# Autodesk Inventor assembly: Wheels_hubs
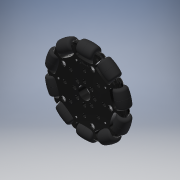
[picture p0: Inventor's stored thumbnail of the model, 180x180]
Saved by Autodesk Inventor 2019 (Build 230136000, 136)
## iProperties
Created: 2018-12-27
Part Number: Wheels_hubs
Document SubType Name: Assembly
Designer: Ashley
Author: Ashley
## Documents named in this file (3)
- C:\Users\mrhftc\repositories\design\inventor\2018-2019\Body Assemblies\Wheels_hubs.iam
- C:\Users\mrhftc\repositories\design\inventor\Imported Components\goBilda\CampingHub\ClampingHub assembly.iam
- C:\Users\mrhftc\repositories\design\inventor\Imported Components\goBilda\Omni Wheel 96mmD\Omni Wheel 96mmD.iam
## Components (2 placed, 2 different names)
1. ClampingHub assembly:1 [sub-assembly] — Insert:1, Mate:1, Mate:2, Mate:3, Mate:4
2. Omni Wheel 96mmD:1 [sub-assembly] — Insert:1, Mate:1, Mate:2, Mate:3, Mate:4
## Relationships (5: Mate 4, Insert 1)
- Insert:1: ClampingHub assembly:1 ↔ Omni Wheel 96mmD:1
- Mate:1: ClampingHub assembly:1 ↔ Omni Wheel 96mmD:1
- Mate:2: ClampingHub assembly:1 ↔ Omni Wheel 96mmD:1
- Mate:3: ClampingHub assembly:1 ↔ Omni Wheel 96mmD:1
- Mate:4: ClampingHub assembly:1 ↔ Omni Wheel 96mmD:1
